# Autodesk Inventor assembly: solenoid
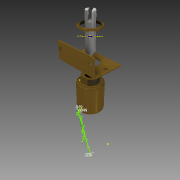
[picture p0: Inventor's stored thumbnail of the model, 180x180]
Saved by Autodesk Inventor 2014 (Build 180170000, 170)
## iProperties
Created: 2013-07-22
Part Number: solenoid
Document SubType Name: Assembly
Designer: Saville
Mass: 37.952 g
Surface Area: 342.268 cm^2
Volume: 37.952 cm^3
Density: 1 g/cm^3
Author: Saville
## Documents named in this file (6)
- C:\shotgun\solenoid.iam
- C:\shotgun\solenoid body.ipt
- C:\shotgun\solenoid nut.ipt
- C:\shotgun\washer.ipt
- C:\shotgun\bracket.ipt
- C:\shotgun\solenoid pin.ipt
## Components (5 placed, 5 different names)
1. solenoid body:1 — Mate:1, Mate:2, Mate:3, Mate:4
2. solenoid nut:1 — Mate:1
3. washer:1 — Mate:2
4. bracket:1 — Mate:3
5. solenoid pin:1 — Mate:4
## Relationships (4: Mate 4)
- Mate:1: solenoid body:1 ↔ solenoid nut:1
- Mate:2: solenoid body:1 ↔ washer:1
- Mate:3: solenoid body:1 ↔ bracket:1
- Mate:4: solenoid body:1 ↔ solenoid pin:1
